# Autodesk Inventor assembly: IRB120_3-58_IRC5_rev1
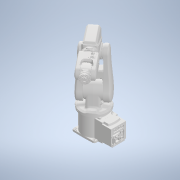
[picture p0: Inventor's stored thumbnail of the model, 180x180]
Saved by Autodesk Inventor 2021 (Build 250183000, 183)
## iProperties
Company: ABB
Created: 2017-02-17
Part Number: IRB120_3-58_IRC5_rev1
Description: STEP AP203
Document SubType Name: Assembly
Designer: mahmo
Sending System: SolidWorks 2014
Preprocessor: SwSTEP 2.0
Title: IRB120_3-58_IRC5_rev1.STEP
Author: ABB
Revision Number: ANY
## Documents named in this file (8)
- D:\new_gripper\IRB120_3-58_irc5_rev01_step_j\IRB120_3-58_irc5_rel1_step_j\STEP Files\IRB120_3-58_IRB5_rev1_STEP_c\IRB120_3-58_IRC5_rev1.iam
- D:\new_gripper\IRB120_3-58_irc5_rev01_step_j\IRB120_3-58_irc5_rel1_step_j\STEP Files\IRB120_3-58_IRB5_rev1_STEP_c\IRB120_3-58_IRC5_Base_rev1.ipt
- D:\new_gripper\IRB120_3-58_irc5_rev01_step_j\IRB120_3-58_irc5_rel1_step_j\STEP Files\IRB120_3-58_IRB5_rev1_STEP_c\IRB120_3-58_IRC5_Link1_rev1.ipt
- D:\new_gripper\IRB120_3-58_irc5_rev01_step_j\IRB120_3-58_irc5_rel1_step_j\STEP Files\IRB120_3-58_IRB5_rev1_STEP_c\IRB120_3-58_IRC5_Link2_rev1.ipt
- D:\new_gripper\IRB120_3-58_irc5_rev01_step_j\IRB120_3-58_irc5_rel1_step_j\STEP Files\IRB120_3-58_IRB5_rev1_STEP_c\IRB120_3-58_IRC5_Link3_rev1.ipt
- D:\new_gripper\IRB120_3-58_irc5_rev01_step_j\IRB120_3-58_irc5_rel1_step_j\STEP Files\IRB120_3-58_IRB5_rev1_STEP_c\IRB120_3-58_IRC5_Link4_rev1.ipt
- D:\new_gripper\IRB120_3-58_irc5_rev01_step_j\IRB120_3-58_irc5_rel1_step_j\STEP Files\IRB120_3-58_IRB5_rev1_STEP_c\IRB120_3-58_IRC5_Link6_rev1.ipt
- D:\new_gripper\IRB120_3-58_irc5_rev01_step_j\IRB120_3-58_irc5_rel1_step_j\STEP Files\IRB120_3-58_IRB5_rev1_STEP_c\IRB120_3-58_IRC5_Link5_rev1.ipt
## Components (7 placed, 7 different names)
1. IRB120_3-58_IRC5_Base_rev1_1 — Mate:3, Mate:4, Angle:1
2. IRB120_3-58_IRC5_Link1_rev1_2 — Mate:3, Mate:4, Mate:5, Mate:6
3. IRB120_3-58_IRC5_Link2_rev1_3 — Mate:1, Mate:2, Mate:5, Mate:6
4. IRB120_3-58_IRC5_Link3_rev1_4 — Mate:1, Mate:2, Mate:7, Mate:8
5. IRB120_3-58_IRC5_Link4_rev1_5 — Mate:7, Mate:8, Mate:9, Mate:10
6. IRB120_3-58_IRC5_Link6_rev1_6 — Mate:11, Mate:12
7. IRB120_3-58_IRC5_Link5_rev1_7 — Mate:9, Mate:10, Mate:11, Mate:12, Angle:1
## Relationships (13: Mate 12, Angle 1)
- Mate:1: IRB120_3-58_IRC5_Link2_rev1_3 ↔ IRB120_3-58_IRC5_Link3_rev1_4
- Mate:2: IRB120_3-58_IRC5_Link2_rev1_3 ↔ IRB120_3-58_IRC5_Link3_rev1_4
- Mate:3: IRB120_3-58_IRC5_Base_rev1_1 ↔ IRB120_3-58_IRC5_Link1_rev1_2
- Mate:4: IRB120_3-58_IRC5_Base_rev1_1 ↔ IRB120_3-58_IRC5_Link1_rev1_2
- Mate:5: IRB120_3-58_IRC5_Link1_rev1_2 ↔ IRB120_3-58_IRC5_Link2_rev1_3
- Mate:6: IRB120_3-58_IRC5_Link1_rev1_2 ↔ IRB120_3-58_IRC5_Link2_rev1_3
- Mate:7: IRB120_3-58_IRC5_Link3_rev1_4 ↔ IRB120_3-58_IRC5_Link4_rev1_5
- Mate:8: IRB120_3-58_IRC5_Link3_rev1_4 ↔ IRB120_3-58_IRC5_Link4_rev1_5
- Mate:9: IRB120_3-58_IRC5_Link4_rev1_5 ↔ IRB120_3-58_IRC5_Link5_rev1_7
- Mate:10: IRB120_3-58_IRC5_Link4_rev1_5 ↔ IRB120_3-58_IRC5_Link5_rev1_7
- Mate:11: IRB120_3-58_IRC5_Link6_rev1_6 ↔ IRB120_3-58_IRC5_Link5_rev1_7
- Mate:12: IRB120_3-58_IRC5_Link6_rev1_6 ↔ IRB120_3-58_IRC5_Link5_rev1_7
- Angle:1 (0 deg): IRB120_3-58_IRC5_Base_rev1_1 ↔ IRB120_3-58_IRC5_Link5_rev1_7
